# Autodesk Inventor assembly: warthog_right_assembly
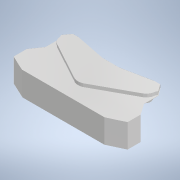
[picture p0: Inventor's stored thumbnail of the model, 180x180]
Saved by Autodesk Inventor 2021 (Build 250183000, 183)
## iProperties
Created: 2020-04-08
Part Number: warthog_right_assembly
Document SubType Name: Assembly
Designer: jules
Author: jules
## Documents named in this file (6)
- C:\Users\jules\Documents\ENSTA Bretagne\2A\UE 4.2 - Simulation des robots mobiles\WARTHOG\Elements de CAO - Fichiers STL-20200408\warthog_right_assembly.iam
- C:\Users\jules\Documents\Inventor\chassis.ipt
- C:\Users\jules\Documents\ENSTA Bretagne\2A\UE 4.2 - Simulation des robots mobiles\WARTHOG\Elements de CAO - Fichiers STL-20200408\Imported Components\rocker\rocker.ipt
- C:\Users\jules\Documents\ENSTA Bretagne\2A\UE 4.2 - Simulation des robots mobiles\WARTHOG\Elements de CAO - Fichiers STL-20200408\Imported Components\wheel\wheel.ipt
- C:\Users\jules\Documents\ENSTA Bretagne\2A\UE 4.2 - Simulation des robots mobiles\WARTHOG\Elements de CAO - Fichiers STL-20200408\Imported Components\bulkhead\bulkhead.ipt
- C:\Users\jules\Documents\ENSTA Bretagne\2A\UE 4.2 - Simulation des robots mobiles\WARTHOG\Elements de CAO - Fichiers STL-20200408\Imported Components\fenders\fenders.ipt
## Components (11 placed, 5 different names)
1. chassis:1 — Mate:9, Mate:10, Flush:1, Flush:2, Flush:3, Flush:4, Mate:11, Flush:5, Flush:6, Mate:12, Flush:7
2. rocker:1 — Mate:3, Mate:4, Mate:7, Mate:8, Mate:10, Flush:2, Flush:3, Mate:14, Flush:10, Flush:11
3. rocker:2 — Mate:1, Mate:2, Mate:5, Mate:6, Mate:9, Flush:1, Flush:4, Mate:15, Flush:8, Flush:9
4. wheel:1 — Mate:1, Mate:5
5. wheel:2 — Mate:2, Mate:6
6. wheel:3 — Mate:3, Mate:8
7. wheel:4 — Mate:4, Mate:7
8. bulkhead:1 — Mate:11, Flush:5, Flush:6, Mate:13
9. bulkhead:2 — Mate:12, Mate:13, Flush:7
10. fenders:1 — Mate:14, Flush:10, Flush:11
11. fenders:2 — Mate:15, Flush:8, Flush:9
## Relationships (26: Mate 15, Flush 11)
- Mate:1: rocker:2 ↔ wheel:1
- Mate:2: rocker:2 ↔ wheel:2
- Mate:3: rocker:1 ↔ wheel:3
- Mate:4: rocker:1 ↔ wheel:4
- Mate:5: rocker:2 ↔ wheel:1
- Mate:6: rocker:2 ↔ wheel:2
- Mate:7: rocker:1 ↔ wheel:4
- Mate:8: rocker:1 ↔ wheel:3
- Mate:9: chassis:1 ↔ rocker:2
- Mate:10: chassis:1 ↔ rocker:1
- Flush:1: chassis:1 ↔ rocker:2
- Flush:2: chassis:1 ↔ rocker:1
- Flush:3 (-6 mm): chassis:1 ↔ rocker:1
- Flush:4 (-6 mm): chassis:1 ↔ rocker:2
- Mate:11: chassis:1 ↔ bulkhead:1
- Flush:5: chassis:1 ↔ bulkhead:1
- Flush:6: chassis:1 ↔ bulkhead:1
- Mate:12: chassis:1 ↔ bulkhead:2
- Mate:13: bulkhead:1 ↔ bulkhead:2
- Flush:7: chassis:1 ↔ bulkhead:2
- Mate:14: rocker:1 ↔ fenders:1
- Mate:15: rocker:2 ↔ fenders:2
- Flush:8: rocker:2 ↔ fenders:2
- Flush:9: rocker:2 ↔ fenders:2
- Flush:10: rocker:1 ↔ fenders:1
- Flush:11: rocker:1 ↔ fenders:1
